# Autodesk Inventor assembly: FullBuildWood
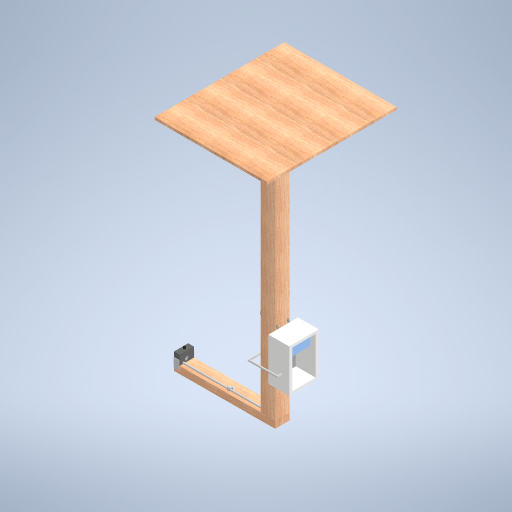
[picture p0: Inventor's stored thumbnail of the model, 512x512]
Saved by Autodesk Inventor 2024.2 (Build 282272000, 272)
## iProperties
Created: 2024-01-23
Part Number: FullBuildWood
Document SubType Name: Assembly
Designer: airso
Author: airso
## Documents named in this file (14)
- C:\Users\airso\OneDrive\Documents\school\2023 Fall\Capstone\Inventor Files\FullBuildWood.iam
- C:\Users\airso\OneDrive\Documents\school\2023 Fall\Capstone\Inventor Files\BottomPost.ipt
- C:\Users\airso\OneDrive\Documents\school\2023 Fall\Capstone\Inventor Files\JunctionBox.ipt
- C:\Users\airso\OneDrive\Documents\school\2023 Fall\Capstone\Inventor Files\TopPost.ipt
- C:\Users\airso\OneDrive\Documents\school\2023 Fall\Capstone\Inventor Files\90294A257_Phillips Flat Head Screws for Wood.ipt
- C:\Users\airso\OneDrive\Documents\school\2023 Fall\Capstone\Inventor Files\BoxMountingMetal.ipt
- C:\Users\airso\OneDrive\Documents\school\2023 Fall\Capstone\Inventor Files\90294A153_Phillips Flat Head Screws for Wood.ipt
- C:\Users\airso\OneDrive\Documents\school\2023 Fall\Capstone\Inventor Files\Wiretube.ipt
- C:\Users\airso\OneDrive\Documents\school\2023 Fall\Capstone\Inventor Files\BendTube.ipt
- C:\Users\airso\OneDrive\Documents\school\2023 Fall\Capstone\Inventor Files\WoodBase.ipt
- C:\Users\airso\OneDrive\Documents\school\2023 Fall\Capstone\Inventor Files\PostBase.ipt
- C:\Users\airso\OneDrive\Documents\school\2023 Fall\Capstone\Inventor Files\Routing Clamp.ipt
- C:\Users\airso\OneDrive\Documents\school\2023 Fall\Capstone\Inventor Files\SensorBoxBraket.ipt
- C:\Users\airso\OneDrive\Documents\school\2023 Fall\Capstone\Inventor Files\sensorbox\Component1.ipt
## Components (37 placed, 13 different names)
1. BottomPost:1 — Mate:2, Flush:1, Flush:2, Mate:3, Flush:7, Mate:4, Mate:5, Mate:6, Mate:7, Mate:12, Mate:13, Mate:14, Mate:15, Flush:8, Flush:9, Flush:10, Flush:11, Mate:32, Mate:34, Mate:35, Mate:37, Mate:38, Mate:40, Mate:42, Mate:43
2. JunctionBox:1 — Mate:3, Flush:7, Mate:8, Mate:9, Mate:10, Mate:11, Mate:39, Mate:41, Flush:27
3. TopPost:1 — Mate:2, Flush:1, Flush:2, Flush:3, Flush:4, Flush:5, Flush:6, Mate:31, Mate:44, Flush:12, Mate:47, Mate:48, Flush:13, Mate:53, Mate:54, Mate:56, Mate:57, Flush:17, Flush:18, Flush:27
4. 90294A257_Phillips Flat Head Screws for Wood:1 — Flush:3
5. 90294A257_Phillips Flat Head Screws for Wood:2 — Flush:4
6. 90294A257_Phillips Flat Head Screws for Wood:3 — Flush:5
7. 90294A257_Phillips Flat Head Screws for Wood:4 — Flush:6
8. BoxMountingMetal:1 — Mate:4, Mate:10, Mate:13, Mate:19
9. BoxMountingMetal:2 — Mate:6, Mate:11, Mate:12, Mate:18
10. BoxMountingMetal:3 — Mate:5, Mate:9, Mate:14, Mate:17
11. BoxMountingMetal:4 — Mate:7, Mate:8, Mate:15, Mate:16
12. 90294A153_Phillips Flat Head Screws for Wood:1 — Mate:16, Flush:11
13. 90294A153_Phillips Flat Head Screws for Wood:2 — Mate:18, Flush:8
14. 90294A153_Phillips Flat Head Screws for Wood:3 — Mate:17, Flush:10
15. 90294A153_Phillips Flat Head Screws for Wood:4 — Mate:19, Flush:9
16. Wiretube:1 — Mate:31, Mate:32, Mate:34, Mate:45, Mate:46
17. BendTube:1 — Mate:39, Mate:40, Mate:41
18. WoodBase:1 — Mate:35, Mate:36
19. PostBase:1 — Mate:36, Mate:37, Mate:38
20. Routing Clamp:1 — Mate:43, Mate:46, Flush:12, Mate:51, Flush:16
21. Routing Clamp:2 — Mate:44, Mate:49, Mate:52, Flush:15
22. Routing Clamp:3 — Mate:42, Mate:45, Mate:50, Flush:14
23. Wiretube:2 — Mate:47, Mate:48, Flush:13, Mate:49
24. 90294A153_Phillips Flat Head Screws for Wood:5 — Mate:50, Flush:14
25. 90294A153_Phillips Flat Head Screws for Wood:6 — Mate:51, Flush:16
26. 90294A153_Phillips Flat Head Screws for Wood:7 — Mate:52, Flush:15
27. SensorBoxBraket:1 — Mate:53, Mate:58, Mate:59, Mate:61, Mate:62, Mate:63, Mate:64, Flush:23, Flush:24, Flush:25, Flush:26
28. SensorBoxBraket:2 — Mate:54, Mate:60, Flush:18, Mate:65, Mate:66, Mate:67, Mate:68, Flush:19, Flush:20, Flush:21, Flush:22
29. Component1:1 — Mate:56, Mate:57, Flush:17, Mate:58, Mate:59, Mate:60
30. 90294A153_Phillips Flat Head Screws for Wood:8 — Mate:63, Flush:25
31. 90294A153_Phillips Flat Head Screws for Wood:9 — Mate:64, Flush:26
32. 90294A153_Phillips Flat Head Screws for Wood:10 — Mate:65, Flush:22
33. 90294A153_Phillips Flat Head Screws for Wood:11 — Mate:62, Flush:24
34. 90294A153_Phillips Flat Head Screws for Wood:12 — Mate:68, Flush:20
35. 90294A153_Phillips Flat Head Screws for Wood:13 — Mate:66, Flush:21
36. 90294A153_Phillips Flat Head Screws for Wood:14 — Mate:61, Flush:23
37. 90294A153_Phillips Flat Head Screws for Wood:15 — Mate:67, Flush:19
## Relationships (81: Mate 54, Flush 27)
- Mate:2: BottomPost:1 ↔ TopPost:1
- Flush:1: BottomPost:1 ↔ TopPost:1
- Flush:2: BottomPost:1 ↔ TopPost:1
- Flush:3 (-2.54 mm): TopPost:1 ↔ 90294A257_Phillips Flat Head Screws for Wood:1
- Flush:4 (-2.54 mm): TopPost:1 ↔ 90294A257_Phillips Flat Head Screws for Wood:2
- Flush:5 (-2.54 mm): TopPost:1 ↔ 90294A257_Phillips Flat Head Screws for Wood:3
- Flush:6 (-2.54 mm): TopPost:1 ↔ 90294A257_Phillips Flat Head Screws for Wood:4
- Mate:3 (6.096 mm): BottomPost:1 ↔ JunctionBox:1
- Flush:7 (-53.975 mm): BottomPost:1 ↔ JunctionBox:1
- Mate:4: BottomPost:1 ↔ BoxMountingMetal:1
- Mate:5: BottomPost:1 ↔ BoxMountingMetal:3
- Mate:6: BottomPost:1 ↔ BoxMountingMetal:2
- Mate:7: BottomPost:1 ↔ BoxMountingMetal:4
- Mate:8: JunctionBox:1 ↔ BoxMountingMetal:4
- Mate:9: JunctionBox:1 ↔ BoxMountingMetal:3
- Mate:10: JunctionBox:1 ↔ BoxMountingMetal:1
- Mate:11: JunctionBox:1 ↔ BoxMountingMetal:2
- Mate:12 (-12.7 mm): BottomPost:1 ↔ BoxMountingMetal:2
- Mate:13 (-12.7 mm): BottomPost:1 ↔ BoxMountingMetal:1
- Mate:14 (-12.7 mm): BottomPost:1 ↔ BoxMountingMetal:3
- Mate:15 (-12.7 mm): BottomPost:1 ↔ BoxMountingMetal:4
- Mate:16: BoxMountingMetal:4 ↔ 90294A153_Phillips Flat Head Screws for Wood:1
- Mate:17: BoxMountingMetal:3 ↔ 90294A153_Phillips Flat Head Screws for Wood:3
- Mate:18: BoxMountingMetal:2 ↔ 90294A153_Phillips Flat Head Screws for Wood:2
- Mate:19: BoxMountingMetal:1 ↔ 90294A153_Phillips Flat Head Screws for Wood:4
- Flush:8 (-2.54 mm): BottomPost:1 ↔ 90294A153_Phillips Flat Head Screws for Wood:2
- Flush:9 (-2.54 mm): BottomPost:1 ↔ 90294A153_Phillips Flat Head Screws for Wood:4
- Flush:10 (-2.54 mm): BottomPost:1 ↔ 90294A153_Phillips Flat Head Screws for Wood:3
- Flush:11 (-2.54 mm): BottomPost:1 ↔ 90294A153_Phillips Flat Head Screws for Wood:1
- Mate:31: TopPost:1 ↔ Wiretube:1
- Mate:32 (6.35 mm): BottomPost:1 ↔ Wiretube:1
- Mate:34 (76.2 mm): BottomPost:1 ↔ Wiretube:1
- Mate:35: BottomPost:1 ↔ WoodBase:1
- Mate:36: WoodBase:1 ↔ PostBase:1
- Mate:37: BottomPost:1 ↔ PostBase:1
- Mate:38: BottomPost:1 ↔ PostBase:1
- Mate:39: JunctionBox:1 ↔ BendTube:1
- Mate:40 (6.35 mm): BottomPost:1 ↔ BendTube:1
- Mate:41 (-101.6 mm): JunctionBox:1 ↔ BendTube:1
- Mate:42: BottomPost:1 ↔ Routing Clamp:3
- Mate:43: BottomPost:1 ↔ Routing Clamp:1
- Mate:44: TopPost:1 ↔ Routing Clamp:2
- Mate:45 (4.572 mm): Wiretube:1 ↔ Routing Clamp:3
- Mate:46 (4.572 mm): Wiretube:1 ↔ Routing Clamp:1
- Flush:12 (-50.8 mm): TopPost:1 ↔ Routing Clamp:1
- Mate:47 (6.35 mm): TopPost:1 ↔ Wiretube:2
- Mate:48 (76.2 mm): TopPost:1 ↔ Wiretube:2
- Flush:13 (38.1 mm): TopPost:1 ↔ Wiretube:2
- Mate:49 (4.572 mm): Routing Clamp:2 ↔ Wiretube:2
- Mate:50: Routing Clamp:3 ↔ 90294A153_Phillips Flat Head Screws for Wood:5
- Flush:14 (-1.27 mm): Routing Clamp:3 ↔ 90294A153_Phillips Flat Head Screws for Wood:5
- Mate:51: Routing Clamp:1 ↔ 90294A153_Phillips Flat Head Screws for Wood:6
- Mate:52: Routing Clamp:2 ↔ 90294A153_Phillips Flat Head Screws for Wood:7
- Flush:15 (-1.27 mm): Routing Clamp:2 ↔ 90294A153_Phillips Flat Head Screws for Wood:7
- Flush:16 (-1.27 mm): Routing Clamp:1 ↔ 90294A153_Phillips Flat Head Screws for Wood:6
- Mate:53: TopPost:1 ↔ SensorBoxBraket:1
- Mate:54: TopPost:1 ↔ SensorBoxBraket:2
- Mate:56: TopPost:1 ↔ Component1:1
- Mate:57: TopPost:1 ↔ Component1:1
- Flush:17: TopPost:1 ↔ Component1:1
- Mate:58 (93.98 mm): SensorBoxBraket:1 ↔ Component1:1
- Mate:59: SensorBoxBraket:1 ↔ Component1:1
- Mate:60 (34.036 mm): SensorBoxBraket:2 ↔ Component1:1
- Flush:18: TopPost:1 ↔ SensorBoxBraket:2
- Mate:61: SensorBoxBraket:1 ↔ 90294A153_Phillips Flat Head Screws for Wood:14
- Mate:62: SensorBoxBraket:1 ↔ 90294A153_Phillips Flat Head Screws for Wood:11
- Mate:63: SensorBoxBraket:1 ↔ 90294A153_Phillips Flat Head Screws for Wood:8
- Mate:64: SensorBoxBraket:1 ↔ 90294A153_Phillips Flat Head Screws for Wood:9
- Mate:65: SensorBoxBraket:2 ↔ 90294A153_Phillips Flat Head Screws for Wood:10
- Mate:66: SensorBoxBraket:2 ↔ 90294A153_Phillips Flat Head Screws for Wood:13
- Mate:67: SensorBoxBraket:2 ↔ 90294A153_Phillips Flat Head Screws for Wood:15
- Mate:68: SensorBoxBraket:2 ↔ 90294A153_Phillips Flat Head Screws for Wood:12
- Flush:19 (-1.27 mm): SensorBoxBraket:2 ↔ 90294A153_Phillips Flat Head Screws for Wood:15
- Flush:20 (-1.27 mm): SensorBoxBraket:2 ↔ 90294A153_Phillips Flat Head Screws for Wood:12
- Flush:21 (-1.27 mm): SensorBoxBraket:2 ↔ 90294A153_Phillips Flat Head Screws for Wood:13
- Flush:22 (-1.27 mm): SensorBoxBraket:2 ↔ 90294A153_Phillips Flat Head Screws for Wood:10
- Flush:23 (-1.27 mm): SensorBoxBraket:1 ↔ 90294A153_Phillips Flat Head Screws for Wood:14
- Flush:24 (-1.27 mm): SensorBoxBraket:1 ↔ 90294A153_Phillips Flat Head Screws for Wood:11
- Flush:25 (-1.27 mm): SensorBoxBraket:1 ↔ 90294A153_Phillips Flat Head Screws for Wood:8
- Flush:26 (-1.27 mm): SensorBoxBraket:1 ↔ 90294A153_Phillips Flat Head Screws for Wood:9
- Flush:27 (304.8 mm): JunctionBox:1 ↔ TopPost:1
